# Autodesk Inventor assembly: base assembly
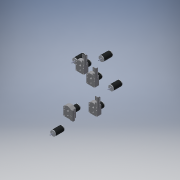
[picture p0: Inventor's stored thumbnail of the model, 180x180]
Saved by Autodesk Inventor 2016 SP2 (Build 200236200, 236)
## iProperties
Created: 2018-01-18
Part Number: base assembly
Document SubType Name: Assembly
Designer: CAD
Author: CAD
## Documents named in this file (4)
- C:\Users\CAD\Documents\GitHub\FIRST-ROBOTICS-2018-5436-CAD\Chassis\base assembly.iam
- C:\Users\CAD\Documents\GitHub\FIRST-ROBOTICS-2018-5436-CAD\Chassis\CIM Motor.ipt
- C:\Users\CAD\Documents\GitHub\FIRST-ROBOTICS-2018-5436-CAD\Chassis\Transmission box.ipt
- C:\Users\CAD\Documents\GitHub\FIRST-ROBOTICS-2018-5436-CAD\Chassis\Transmission bracket.ipt
## Components (16 placed, 3 different names)
1. CIM Motor:1
2. Transmission box:1 — Insert:1
3. Transmission bracket:1 — Insert:1
4. CIM Motor:2
5. Transmission box:2
6. Transmission bracket:2
7. CIM Motor:3
8. Transmission box:3
9. Transmission bracket:3
10. CIM Motor:4
11. Transmission box:4
12. Transmission bracket:4
13. CIM Motor:5
14. CIM Motor:6
15. CIM Motor:7
16. CIM Motor:8
## Relationships (1: Insert 1)
- Insert:1: Transmission box:1 ↔ Transmission bracket:1
